# Autodesk Inventor assembly: PulleySystem
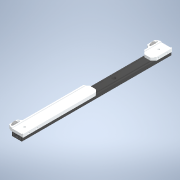
[picture p0: Inventor's stored thumbnail of the model, 180x180]
Saved by Autodesk Inventor 2020 (Build 240168000, 168)
## iProperties
Created: 2020-02-03
Part Number: PulleySystem
Document SubType Name: Assembly
Designer: maple
Author: maple
## Documents named in this file (5)
- C:\Users\maple\Documents\GitHub\CAD\Robotics 2019-2020\PulleySystem\PulleySystem.iam
- C:\Users\maple\Documents\GitHub\CAD\Robotics 2019-2020\PulleySystem\8x20x300mm-v2.ipt
- C:\Users\maple\Documents\GitHub\CAD\Robotics 2019-2020\PulleySystem\3D-Print-Insert-Full-Multibody.ipt
- C:\Users\maple\Documents\GitHub\CAD\Robotics 2019-2020\PulleySystem\3D-Print-Insert-Partial.ipt
- C:\Users\maple\Documents\GitHub\CAD\Robotics 2019-2020\PulleySystem\REV-41-1368.ipt
## Components (5 placed, 4 different names)
1. 8x20x300mm-v2:1 — Rotational:1, Rotational:2
2. 3D-Print-Insert-Full-Multibody:1 — Rotational:1, Rotational:3
3. 3D-Print-Insert-Partial:1 — Rotational:2, Rotational:4
4. REV-41-1368:1 — Rotational:4
5. REV-41-1368:2 — Rotational:3
## Relationships (4: RevoluteJoint 4)
- Rotational:1 [RevoluteJoint]: 8x20x300mm-v2:1 ↔ 3D-Print-Insert-Full-Multibody:1
- Rotational:2 [RevoluteJoint]: 8x20x300mm-v2:1 ↔ 3D-Print-Insert-Partial:1
- Rotational:3 [RevoluteJoint] (-4.7625 mm): 3D-Print-Insert-Full-Multibody:1 ↔ REV-41-1368:2
- Rotational:4 [RevoluteJoint]: 3D-Print-Insert-Partial:1 ↔ REV-41-1368:1
